# Autodesk Inventor assembly: Zespół1
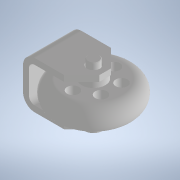
[picture p0: Inventor's stored thumbnail of the model, 180x180]
Saved by Autodesk Inventor 2021 (Build 250183000, 183)
## iProperties
Created: 2021-05-26
Part Number: Zespół1
Document SubType Name: Assembly
Designer: DESKTOP-12
Author: DESKTOP-12
## Documents named in this file (5)
- E:\Studia\S08 (06)\Projektowanie wspomagane komputerowo P\Inventor\Zespół1.iam
- E:\Studia\S08 (06)\Projektowanie wspomagane komputerowo P\Inventor\Blacha.ipt
- E:\Studia\S08 (06)\Projektowanie wspomagane komputerowo P\Inventor\Koło.ipt
- E:\Studia\S08 (06)\Projektowanie wspomagane komputerowo P\Inventor\Trzpień.ipt
- C:\Users\DESKTOP-12\Documents\Inventor\Content Center Files\R2021\pl-PL\ISO 7434(2)\ISO 7434 - M3 x 8ISO.ipt
## Components (4 placed, 4 different names)
1. Blacha:1 — Zestawiające:1, Zestawiające:2, Wstawiające:1
2. Koło:1 — Zestawiające:1, Zestawiające:2
3. Trzpień:1 — Wstawiające:1, Wstawiające:2
4. ISO 7434 M3x8:1 — Wstawiające:2
## Relationships (4: Mate 2, Insert 2)
- Zestawiające:1 [Mate]: Blacha:1 ↔ Koło:1
- Zestawiające:2 [Mate]: Blacha:1 ↔ Koło:1
- Wstawiające:1 [Insert]: Blacha:1 ↔ Trzpień:1
- Wstawiające:2 [Insert] (-6 mm): Trzpień:1 ↔ ISO 7434 M3x8:1
